# Autodesk Inventor assembly: doorLockAssembly_V5
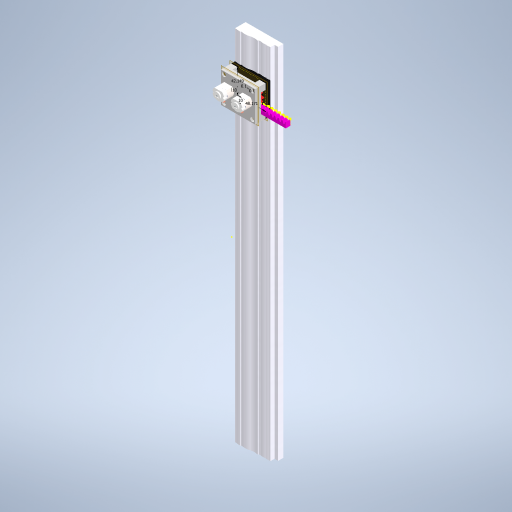
[picture p0: Inventor's stored thumbnail of the model, 512x512]
Saved by Autodesk Inventor 2023 (Build 270158000, 158)
## iProperties
Created: 2023-03-11
Part Number: doorLockAssembly_V5
Document SubType Name: Assembly
Designer: shrey
Author: shrey
## Documents named in this file (8)
- D:\Inventor Projects\Door Lock\V5\doorLockAssembly_V5.iam
- D:\Inventor Projects\Door Lock\V4\moulding.ipt
- D:\Inventor Projects\Door Lock\V4\pinion_V4.ipt
- D:\Inventor Projects\Door Lock\V4\screw.ipt
- D:\Inventor Projects\Door Lock\motor.ipt
- D:\Inventor Projects\Door Lock\V5\house_V5.ipt
- D:\Inventor Projects\Door Lock\V5\housePlate_V5.ipt
- D:\Inventor Projects\Door Lock\V3\rack_V3.ipt
## Components (9 placed, 7 different names)
1. moulding:1 — Mate:1, Flush:1, Mate:2, Flush:5
2. pinion_V4:1 — Mate:6, Flush:4, Mate:11
3. screw:1 — Mate:12, Mate:13
4. motor:1 — Mate:6, Flush:4
5. motor:2 — Flush:3, Mate:5
6. house_V5:1 — Mate:3, Mate:4, Flush:2, Flush:10, Mate:13
7. pinion_V4:2 — Flush:3, Mate:5, Mate:10
8. housePlate_V5:1 — Mate:7, Mate:8, Flush:6, Flush:7, Flush:8, Mate:9, Flush:9, Mate:10, Mate:11, Flush:10, Mate:12
9. rack_V3:1 — Flush:8, Mate:9, Flush:9
## Relationships (23: Mate 13, Flush 10)
- Mate:1: moulding:1
- Flush:1: moulding:1
- Mate:2: moulding:1
- Mate:3: house_V5:1
- Mate:4: house_V5:1
- Flush:2: house_V5:1
- Flush:3: motor:2 ↔ pinion_V4:2
- Mate:5: motor:2 ↔ pinion_V4:2
- Mate:6: pinion_V4:1 ↔ motor:1
- Flush:4: pinion_V4:1 ↔ motor:1
- Flush:5 (-18.749 mm): moulding:1
- Mate:7: housePlate_V5:1
- Mate:8: housePlate_V5:1
- Flush:6: housePlate_V5:1
- Flush:7: housePlate_V5:1
- Flush:8 (-10.15 mm): housePlate_V5:1 ↔ rack_V3:1
- Mate:9: housePlate_V5:1 ↔ rack_V3:1
- Flush:9: housePlate_V5:1 ↔ rack_V3:1
- Mate:10: pinion_V4:2 ↔ housePlate_V5:1
- Mate:11: pinion_V4:1 ↔ housePlate_V5:1
- Flush:10: house_V5:1 ↔ housePlate_V5:1
- Mate:12 (-3 mm): screw:1 ↔ housePlate_V5:1
- Mate:13: screw:1 ↔ house_V5:1
